# Autodesk Inventor assembly: RT_FRM_A_004_ElectricalFrame
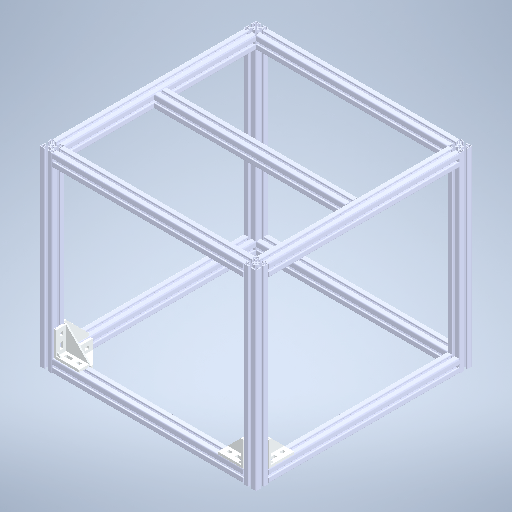
[picture p0: Inventor's stored thumbnail of the model, 512x512]
Saved by Autodesk Inventor 2025.3 (Build 293356000, 356)
## iProperties
Created: 2026-05-11
Part Number: RT_FRM_A_004_ElectricalFrame
Document SubType Name: Assembly
Designer: louis
Author: louis
## Documents named in this file (9)
- C:\Users\louis\OneDrive\Desktop\R_Trident\02_CAD\04_Subassemblies\RT_FRM_A_004_ElectricalFrame.iam
- C:\Users\louis\OneDrive\Desktop\R_Trident\02_CAD\01_Standard_Parts\Aluminium_Extrusions\4040x600_3619_20251007144627_4040.ipt
- C:\Users\louis\OneDrive\Desktop\R_Trident\02_CAD\01_Standard_Parts\3532_20210408113519_4080L + cover\3532_20210408113519_4080L + cover.iam
- C:\Users\louis\OneDrive\Desktop\R_Trident\02_CAD\04_Subassemblies\RT_FRM_A_004_ElectricalFrame\AIP\FEA\fg20fls1s.fins
- C:\Users\louis\OneDrive\Desktop\R_Trident\02_CAD\04_Subassemblies\RT_FRM_A_004_ElectricalFrame\AIP\FEA\fg20fls1s.fsat
- C:\Users\louis\OneDrive\Desktop\R_Trident\02_CAD\04_Subassemblies\RT_FRM_A_004_ElectricalFrame\AIP\FEA\fg20fls1s.ftes
- C:\Users\louis\OneDrive\Desktop\R_Trident\02_CAD\04_Subassemblies\RT_FRM_A_004_ElectricalFrame\AIP\FEA\fg20fls1s.fwiz
- C:\Users\louis\OneDrive\Desktop\R_Trident\02_CAD\04_Subassemblies\RT_FRM_A_004_ElectricalFrame\AIP\FEA\fg20fls68.fmsh
- C:\Users\louis\OneDrive\Desktop\R_Trident\02_CAD\04_Subassemblies\RT_FRM_A_004_ElectricalFrame\AIP\FEA\fg20fls69.fres
## Components (19 placed, 2 different names)
1. 4040x600_3619_20251007144627_4040:1 — Symmetry:1, Flush:43, Flush:46, Flush:47, Mate:36
2. 4040x600_3619_20251007144627_4040:2 — Mate:15, Flush:30, Symmetry:2, Symmetry:3, Flush:41, Flush:42, Flush:44, Mate:35
3. 4040x600_3619_20251007144627_4040:3 — Mate:14, Flush:29, Symmetry:3, Flush:45, Flush:52, Mate:29, Mate:30
4. 4040x600_3619_20251007144627_4040:4 — Symmetry:1, Flush:39, Flush:40, Flush:53, Flush:54, Mate:28
5. 4040x600_3619_20251007144627_4040:5 — Flush:35, Mate:19, Flush:36, Mate:22, Mate:31, Mate:32, Flush:60, Flush:62
6. 4040x600_3619_20251007144627_4040:6 — Symmetry:2, Flush:38, Mate:26, Mate:27, Flush:48, Flush:50, Flush:58, Flush:59, Mate:34
7. 4040x600_3619_20251007144627_4040:7 — Mate:18, Mate:21, Mate:23, Mate:25, Flush:51, Flush:56, Flush:57, Mate:31, Flush:61, Mate:33, Flush:64
8. 4040x600_3619_20251007144627_4040:8 — Flush:49, Flush:55, Mate:32, Mate:41
9. 4040x600_3619_20251007144627_4040:9 — Mate:14, Mate:15, Flush:29, Flush:30, Flush:31
10. 3532_20210408113519_4080L + cover:1 [sub-assembly] — Mate:18, Mate:39, Flush:64
11. 3532_20210408113519_4080L + cover:2 [sub-assembly] — Flush:35, Mate:19, Mate:40
12. 3532_20210408113519_4080L + cover:3 [sub-assembly] — Mate:21, Flush:36, Mate:22
13. 3532_20210408113519_4080L + cover:4 [sub-assembly] — Mate:23, Flush:63, Mate:38
14. 3532_20210408113519_4080L + cover:5 [sub-assembly] — Mate:27, Mate:37, Flush:65
15. 3532_20210408113519_4080L + cover:6 [sub-assembly] — Mate:25, Flush:38, Mate:26
16. 4040x600_3619_20251007144627_4040:10 — Flush:39, Flush:40, Flush:41, Flush:48, Flush:49, Flush:59, Mate:41
17. 4040x600_3619_20251007144627_4040:11 — Flush:42, Flush:43, Flush:44, Flush:50, Flush:51, Flush:57, Flush:58, Mate:34, Mate:35, Mate:36, Mate:37, Flush:63, Mate:38, Flush:65
18. 4040x600_3619_20251007144627_4040:12 — Flush:52, Flush:53, Flush:54, Mate:28, Flush:55, Mate:30
19. 4040x600_3619_20251007144627_4040:13 — Flush:45, Flush:46, Flush:47, Flush:56, Mate:29, Flush:60, Flush:61, Mate:33, Flush:62, Mate:39, Mate:40
## Relationships (63: Flush 35, Mate 25, Symmetry 3)
- Mate:14: 4040x600_3619_20251007144627_4040:3 ↔ 4040x600_3619_20251007144627_4040:9
- Mate:15: 4040x600_3619_20251007144627_4040:2 ↔ 4040x600_3619_20251007144627_4040:9
- Flush:29: 4040x600_3619_20251007144627_4040:3 ↔ 4040x600_3619_20251007144627_4040:9
- Flush:30: 4040x600_3619_20251007144627_4040:2 ↔ 4040x600_3619_20251007144627_4040:9
- Symmetry:1: 4040x600_3619_20251007144627_4040:1 ↔ 4040x600_3619_20251007144627_4040:4
- Symmetry:2: 4040x600_3619_20251007144627_4040:2 ↔ 4040x600_3619_20251007144627_4040:6
- Flush:31: 4040x600_3619_20251007144627_4040:9
- Flush:32
- Flush:33
- Symmetry:3: 4040x600_3619_20251007144627_4040:2 ↔ 4040x600_3619_20251007144627_4040:3
- Mate:16
- Mate:18: 4040x600_3619_20251007144627_4040:7 ↔ 3532_20210408113519_4080L + cover:1
- Flush:35: 4040x600_3619_20251007144627_4040:5 ↔ 3532_20210408113519_4080L + cover:2
- Mate:19: 4040x600_3619_20251007144627_4040:5 ↔ 3532_20210408113519_4080L + cover:2
- Mate:21: 4040x600_3619_20251007144627_4040:7 ↔ 3532_20210408113519_4080L + cover:3
- Flush:36: 4040x600_3619_20251007144627_4040:5 ↔ 3532_20210408113519_4080L + cover:3
- Mate:22: 4040x600_3619_20251007144627_4040:5 ↔ 3532_20210408113519_4080L + cover:3
- Mate:23: 4040x600_3619_20251007144627_4040:7 ↔ 3532_20210408113519_4080L + cover:4
- Mate:25: 4040x600_3619_20251007144627_4040:7 ↔ 3532_20210408113519_4080L + cover:6
- Flush:38: 4040x600_3619_20251007144627_4040:6 ↔ 3532_20210408113519_4080L + cover:6
- Mate:26: 4040x600_3619_20251007144627_4040:6 ↔ 3532_20210408113519_4080L + cover:6
- Mate:27: 4040x600_3619_20251007144627_4040:6 ↔ 3532_20210408113519_4080L + cover:5
- Flush:39: 4040x600_3619_20251007144627_4040:4 ↔ 4040x600_3619_20251007144627_4040:10
- Flush:40: 4040x600_3619_20251007144627_4040:4 ↔ 4040x600_3619_20251007144627_4040:10
- Flush:41: 4040x600_3619_20251007144627_4040:2 ↔ 4040x600_3619_20251007144627_4040:10
- Flush:42: 4040x600_3619_20251007144627_4040:2 ↔ 4040x600_3619_20251007144627_4040:11
- Flush:43: 4040x600_3619_20251007144627_4040:1 ↔ 4040x600_3619_20251007144627_4040:11
- Flush:44: 4040x600_3619_20251007144627_4040:2 ↔ 4040x600_3619_20251007144627_4040:11
- Flush:45: 4040x600_3619_20251007144627_4040:3 ↔ 4040x600_3619_20251007144627_4040:13
- Flush:46: 4040x600_3619_20251007144627_4040:1 ↔ 4040x600_3619_20251007144627_4040:13
- Flush:47: 4040x600_3619_20251007144627_4040:1 ↔ 4040x600_3619_20251007144627_4040:13
- Flush:48: 4040x600_3619_20251007144627_4040:6 ↔ 4040x600_3619_20251007144627_4040:10
- Flush:49: 4040x600_3619_20251007144627_4040:8 ↔ 4040x600_3619_20251007144627_4040:10
- Flush:50: 4040x600_3619_20251007144627_4040:6 ↔ 4040x600_3619_20251007144627_4040:11
- Flush:51: 4040x600_3619_20251007144627_4040:7 ↔ 4040x600_3619_20251007144627_4040:11
- Flush:52: 4040x600_3619_20251007144627_4040:3 ↔ 4040x600_3619_20251007144627_4040:12
- Flush:53: 4040x600_3619_20251007144627_4040:4 ↔ 4040x600_3619_20251007144627_4040:12
- Flush:54: 4040x600_3619_20251007144627_4040:4 ↔ 4040x600_3619_20251007144627_4040:12
- Mate:28: 4040x600_3619_20251007144627_4040:4 ↔ 4040x600_3619_20251007144627_4040:12
- Flush:55: 4040x600_3619_20251007144627_4040:8 ↔ 4040x600_3619_20251007144627_4040:12
- Flush:56: 4040x600_3619_20251007144627_4040:7 ↔ 4040x600_3619_20251007144627_4040:13
- Flush:57: 4040x600_3619_20251007144627_4040:7 ↔ 4040x600_3619_20251007144627_4040:11
- Flush:58: 4040x600_3619_20251007144627_4040:6 ↔ 4040x600_3619_20251007144627_4040:11
- Flush:59: 4040x600_3619_20251007144627_4040:6 ↔ 4040x600_3619_20251007144627_4040:10
- Mate:29: 4040x600_3619_20251007144627_4040:3 ↔ 4040x600_3619_20251007144627_4040:13
- Mate:30: 4040x600_3619_20251007144627_4040:3 ↔ 4040x600_3619_20251007144627_4040:12
- Mate:31: 4040x600_3619_20251007144627_4040:5 ↔ 4040x600_3619_20251007144627_4040:7
- Mate:32: 4040x600_3619_20251007144627_4040:5 ↔ 4040x600_3619_20251007144627_4040:8
- Flush:60: 4040x600_3619_20251007144627_4040:5 ↔ 4040x600_3619_20251007144627_4040:13
- Flush:61: 4040x600_3619_20251007144627_4040:7 ↔ 4040x600_3619_20251007144627_4040:13
- Mate:33: 4040x600_3619_20251007144627_4040:7 ↔ 4040x600_3619_20251007144627_4040:13
- Mate:34: 4040x600_3619_20251007144627_4040:6 ↔ 4040x600_3619_20251007144627_4040:11
- Mate:35: 4040x600_3619_20251007144627_4040:2 ↔ 4040x600_3619_20251007144627_4040:11
- Flush:62: 4040x600_3619_20251007144627_4040:5 ↔ 4040x600_3619_20251007144627_4040:13
- Mate:36: 4040x600_3619_20251007144627_4040:1 ↔ 4040x600_3619_20251007144627_4040:11
- Mate:37: 3532_20210408113519_4080L + cover:5 ↔ 4040x600_3619_20251007144627_4040:11
- Flush:63: 3532_20210408113519_4080L + cover:4 ↔ 4040x600_3619_20251007144627_4040:11
- Mate:38: 3532_20210408113519_4080L + cover:4 ↔ 4040x600_3619_20251007144627_4040:11
- Mate:39: 3532_20210408113519_4080L + cover:1 ↔ 4040x600_3619_20251007144627_4040:13
- Flush:64: 4040x600_3619_20251007144627_4040:7 ↔ 3532_20210408113519_4080L + cover:1
- Mate:40: 3532_20210408113519_4080L + cover:2 ↔ 4040x600_3619_20251007144627_4040:13
- Flush:65: 3532_20210408113519_4080L + cover:5 ↔ 4040x600_3619_20251007144627_4040:11
- Mate:41: 4040x600_3619_20251007144627_4040:8 ↔ 4040x600_3619_20251007144627_4040:10
## Named parameters: sa_0 = 10000, sa_1 = 20000
note: some values were not read from the file. Shown as the stored number, unit unknown: "sa_0", "sa_1".
